# Autodesk Inventor assembly: PA2
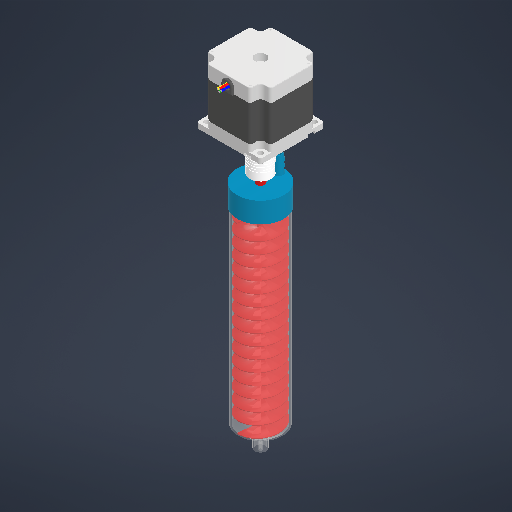
[picture p0: Inventor's stored thumbnail of the model, 512x512]
Saved by Autodesk Inventor 2027 (Build 310192060, 192F)
## iProperties
Created: 2026-08-20
Part Number: PA2
Document SubType Name: Assembly
Designer: trtrn
Author: trtrn
## Documents named in this file (6)
- G:\My Drive\Project\GLUE01\Cad\PA2.iam
- G:\My Drive\Project\GLUE01\Cad\xilanh.ipt
- G:\My Drive\Project\GLUE01\Cad\auger.ipt
- C:\Users\trtrn\OneDrive\Desktop\5mm to 8mm flexible shaft coupler\5mm to 8mm flexible shaft coupler.ipt
- G:\My Drive\Project\GLUE01\Cad\Cap.ipt
- G:\My Drive\Project\GLUE01\Cad\nema23_57byg201\nema23_57byg201.ipt
## Components (5 placed, 5 different names)
1. xilanh:1 — Mate:1, Mate:2, Mate:3
2. auger:1 — Mate:1, Mate:4
3. 5mm to 8mm flexible shaft coupler:1 — Mate:4, Mate:5
4. Cap:1 — Mate:2, Mate:3
5. nema23_57byg201:1 — Mate:5
## Relationships (5: Mate 5)
- Mate:1: xilanh:1 ↔ auger:1
- Mate:2: xilanh:1 ↔ Cap:1
- Mate:3: xilanh:1 ↔ Cap:1
- Mate:4: auger:1 ↔ 5mm to 8mm flexible shaft coupler:1
- Mate:5: 5mm to 8mm flexible shaft coupler:1 ↔ nema23_57byg201:1
